# Autodesk Inventor assembly: muneca
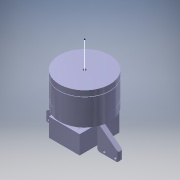
[picture p0: Inventor's stored thumbnail of the model, 180x180]
Saved by Autodesk Inventor 2018 (Build 220112000, 112)
## iProperties
Created: 2018-06-01
Part Number: muneca
Document SubType Name: Assembly
Designer: vigus
Author: vigus
## Documents named in this file (5)
- C:\Users\vigus\Documents\gihug\hecatonquiros\cad_models\accesories\muneca.iam
- C:\Users\vigus\Documents\dji f550\muneca_rodamientos.ipt
- C:\Users\vigus\Documents\dji f550\mun2muneca_rodamientos_1.ipt
- C:\Users\vigus\Documents\dji f550\mun3muneca_rodamiento_2.ipt
- C:\Users\vigus\Documents\dji f550\mun4muneca_rodamiento_3.ipt
## Components (4 placed, 4 different names)
1. muneca_rodamientos:1 — Mate:1, Mate:2, Mate:3, Mate:4
2. mun2muneca_rodamientos_1:1 — Mate:1, Mate:3, Mate:5, Mate:6
3. mun3muneca_rodamiento_2:1 — Mate:2, Mate:4
4. mun4muneca_rodamiento_3:1 — Mate:5, Mate:6
## Relationships (6: Mate 6)
- Mate:1: muneca_rodamientos:1 ↔ mun2muneca_rodamientos_1:1
- Mate:2: muneca_rodamientos:1 ↔ mun3muneca_rodamiento_2:1
- Mate:3: muneca_rodamientos:1 ↔ mun2muneca_rodamientos_1:1
- Mate:4: muneca_rodamientos:1 ↔ mun3muneca_rodamiento_2:1
- Mate:5: mun2muneca_rodamientos_1:1 ↔ mun4muneca_rodamiento_3:1
- Mate:6: mun2muneca_rodamientos_1:1 ↔ mun4muneca_rodamiento_3:1
